# Autodesk Inventor assembly: Agri robot new
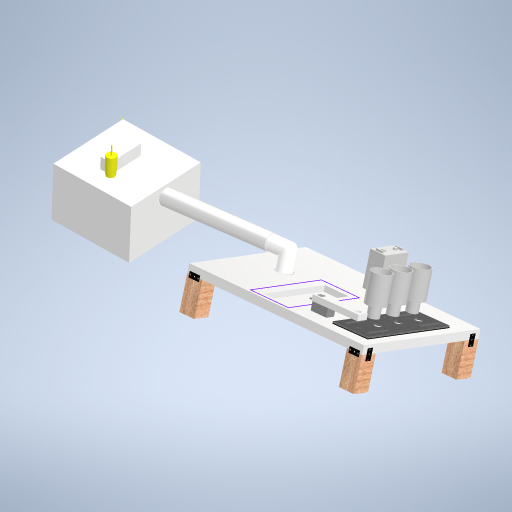
[picture p0: Inventor's stored thumbnail of the model, 512x512]
Saved by Autodesk Inventor 2023 (Build 270158000, 158)
## iProperties
Created: 2022-06-23
Part Number: Agri robot new
Document SubType Name: Assembly
Designer: Shivan
Author: Shivan
## Documents named in this file (14)
- C:\Users\anush\Downloads\Agri robot new.iam
- C:\Users\anush\Downloads\NEW FOLDER\stand.ipt
- C:\Users\anush\Downloads\NEW FOLDER\Sliding Plate.ipt
- C:\Users\anush\Downloads\NEW FOLDER\expo arm.ipt
- C:\Users\anush\Downloads\NEW FOLDER\battery.ipt
- C:\Users\anush\Downloads\NEW FOLDER\Servo motor.ipt
- C:\Users\anush\Downloads\NEW FOLDER\main base new edited new.ipt
- C:\Users\anush\Downloads\NEW FOLDER\new seed container (1).ipt
- C:\Users\anush\Downloads\NEW FOLDER\water tank 1 (1).ipt
- C:\Users\anush\Downloads\NEW FOLDER\pump.ipt
- C:\Users\anush\Downloads\NEW FOLDER\sprayer (1).ipt
- C:\Users\anush\Downloads\NEW FOLDER\L joint.ipt
- C:\Users\anush\Downloads\NEW FOLDER\pipe 1 (1).ipt
- C:\Users\anush\Downloads\NEW FOLDER\clamp.ipt
## Components (25 placed, 13 different names)
1. stand:1 — Rigid:1, Rigid:14, Rigid:15
2. stand:2 — Rigid:3, Rigid:16, Rigid:17
3. stand:3 — Rigid:2, Rigid:18, Rigid:19
4. stand:4 — Flush:1, Mate:17, Rigid:6, Rigid:20, Rigid:21
5. Sliding Plate:1 — Mate:6, Mate:12, Rigid:4, Rigid:5, Rigid:8, Rotational:2, Rotational:3
6. expo arm:1 — Mate:6, Mate:12, Rigid:5, Rotational:1
7. battery:1 — Rigid:7
8. Servo motor:1 — Rotational:1
9. main base new edited new:1 — Rigid:1, Rigid:2, Rigid:3, Flush:1, Mate:17, Rigid:4, Rigid:6, Rigid:7, Rotational:4, Rotational:5
10. new seed container (1):1 — Rigid:8
11. new seed container (1):2 — Rotational:2
12. new seed container (1):3 — Rotational:3
13. sprayer (1):1 — Rotational:4
14. water tank 1 (1):2 — Mate:18, Rigid:11
15. L joint:1 — Rotational:5, Rigid:10
16. pipe 1 (1):1 — Rigid:10, Mate:18
17. pump:2 — Rigid:11
18. clamp:5 — Rigid:18
19. clamp:6 — Rigid:19
20. clamp:7 — Rigid:16
21. clamp:8 — Rigid:15
22. clamp:9 — Rigid:17
23. clamp:10 — Rigid:14
24. clamp:11 — Rigid:21
25. clamp:12 — Rigid:20
## Relationships (28: WeldJoint 18, RevoluteJoint 5, Mate 4, Flush 1)
- Mate:6: Sliding Plate:1 ↔ expo arm:1
- Mate:12: Sliding Plate:1 ↔ expo arm:1
- Rigid:1 [WeldJoint]: stand:1 ↔ main base new edited new:1
- Rigid:2 [WeldJoint]: stand:3 ↔ main base new edited new:1
- Rigid:3 [WeldJoint]: stand:2 ↔ main base new edited new:1
- Flush:1: stand:4 ↔ main base new edited new:1
- Mate:17: stand:4 ↔ main base new edited new:1
- Rigid:4 [WeldJoint]: Sliding Plate:1 ↔ main base new edited new:1
- Rigid:5 [WeldJoint]: Sliding Plate:1 ↔ expo arm:1
- Rotational:1 [RevoluteJoint]: expo arm:1 ↔ Servo motor:1
- Rigid:6 [WeldJoint]: stand:4 ↔ main base new edited new:1
- Rigid:7 [WeldJoint]: battery:1 ↔ main base new edited new:1
- Rigid:8 [WeldJoint]: Sliding Plate:1 ↔ new seed container (1):1
- Rotational:2 [RevoluteJoint]: Sliding Plate:1 ↔ new seed container (1):2
- Rotational:3 [RevoluteJoint]: Sliding Plate:1 ↔ new seed container (1):3
- Rotational:4 [RevoluteJoint]: main base new edited new:1 ↔ sprayer (1):1
- Rotational:5 [RevoluteJoint]: main base new edited new:1 ↔ L joint:1
- Rigid:10 [WeldJoint]: L joint:1 ↔ pipe 1 (1):1
- Mate:18: water tank 1 (1):2 ↔ pipe 1 (1):1
- Rigid:11 [WeldJoint]: water tank 1 (1):2 ↔ pump:2
- Rigid:14 [WeldJoint]: stand:1 ↔ clamp:10
- Rigid:15 [WeldJoint]: stand:1 ↔ clamp:8
- Rigid:16 [WeldJoint]: stand:2 ↔ clamp:7
- Rigid:17 [WeldJoint]: stand:2 ↔ clamp:9
- Rigid:18 [WeldJoint]: stand:3 ↔ clamp:5
- Rigid:19 [WeldJoint]: stand:3 ↔ clamp:6
- Rigid:20 [WeldJoint]: stand:4 ↔ clamp:12
- Rigid:21 [WeldJoint]: stand:4 ↔ clamp:11
